# Autodesk Inventor assembly: CL4-100
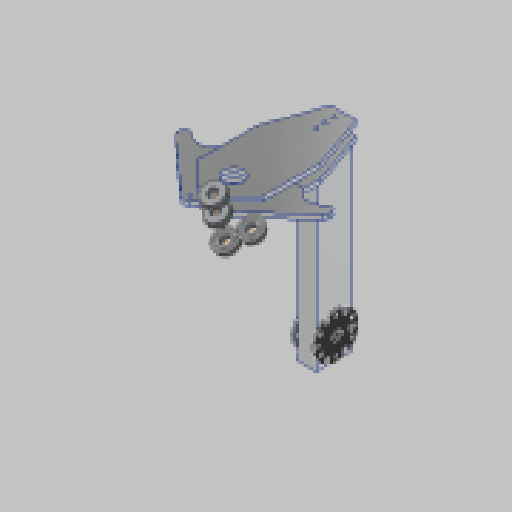
[picture p0: Inventor's stored thumbnail of the model, 512x512]
Saved by Autodesk Inventor 2023.5 (Build 275446000, 446)
## iProperties
Created: 2025-02-04
Part Number: CL4-100
Document SubType Name: Assembly
Designer: brand
Author: brand
## Documents named in this file (11)
- C:\Users\slick\OneDrive\Desktop\2025-ReefScape---CAD\Climber\CL4\CL4-100.iam
- C:\Users\slick\OneDrive\Desktop\2025-ReefScape---CAD\Climber\CL4\CL4-001.ipt
- C:\Users\slick\OneDrive\Desktop\2025-ReefScape---CAD\Climber\CL4\CL4-004.ipt
- C:\Users\slick\OneDrive\Desktop\2025-ReefScape---CAD\Field Items\Full Field\FE-2025\GE-25201.iam
- C:\Users\slick\OneDrive\Desktop\2025-ReefScape---CAD\Climber\CL4\02_Barb Assembly (1)\02_Barb Assembly (1).iam
- C:\Users\slick\OneDrive\Desktop\2025-ReefScape---CAD\Climber\CL4\CL4-005.ipt
- C:\Users\slick\OneDrive\Desktop\2025-ReefScape---CAD\Climber\CL4\CL4-006.ipt
- C:\Users\slick\OneDrive\Desktop\2025-ReefScape---CAD\COMMON PARTS\HUBS\WCP-1388.ipt
- C:\Users\slick\OneDrive\Desktop\2025-ReefScape---CAD\Climber\CL4\CL4-017.ipt
- C:\Users\slick\OneDrive\Desktop\2025-ReefScape---CAD\COMMON PARTS\BEARINGS\0_500_ID_x_1_125_OD_x_0_313_WD_Flanged_Bearing_217-2731.ipt
- C:\Users\slick\OneDrive\Desktop\2025-ReefScape---CAD\Climber\CL4\CL4-022.ipt
## Components (18 placed, 10 different names)
1. CL4-001:1 — Mate:7, Flush:6, Flush:7, Flush:8, Insert:2, Mate:14, Insert:3, Mate:15, Mate:16, Mate:17, Mate:20, Mate:21, Flush:10
2. CL4-005:1 — Flush:8, Flush:9, Mate:8, Mate:17, Insert:4, Insert:8, Insert:11
3. CL4-005:2 — Flush:9, Mate:8, Mate:9, Mate:12, Insert:1, Insert:7, Insert:14
4. CL4-004:1 — Mate:2, Mate:5, Mate:13, Mate:19, Insert:5
5. CL4-004:2 — Mate:2, Mate:5, Mate:9, Mate:12, Mate:13, Mate:18, Insert:6
6. GE-25201:1 [sub-assembly] — Mate:7
7. 02_Barb Assembly (1):1 [sub-assembly] — Flush:6, Flush:7
8. CL4-006:1 — Insert:1, Mate:18, Mate:19
9. WCP-1388:1 — Insert:2, Mate:14
10. WCP-1388:2 — Insert:3, Mate:15
11. CL4-017:1 — Mate:20, Mate:21, Flush:10
12. 0_500_ID_x_1_125_OD_x_0_313_WD_Flanged_Bearing_217-2731:1 — Insert:5, Mate:23
13. 0_500_ID_x_1_125_OD_x_0_313_WD_Flanged_Bearing_217-2731:2 — Insert:6, Mate:22
14. 0_500_ID_x_1_125_OD_x_0_313_WD_Flanged_Bearing_217-2731:3 — Insert:7, Mate:22
15. 0_500_ID_x_1_125_OD_x_0_313_WD_Flanged_Bearing_217-2731:4 — Insert:4, Mate:23
16. CL4-022:1 — Insert:8, Insert:9, Insert:11, Insert:12
17. CL4-022:2 — Insert:9, Insert:10, Insert:12, Insert:13
18. CL4-022:3 — Insert:10, Insert:13, Insert:14
## Relationships (37: Mate 17, Insert 14, Flush 6)
- Mate:2: CL4-004:1 ↔ CL4-004:2
- Mate:5: CL4-004:1 ↔ CL4-004:2
- [Flush]: CL4-001:1 ↔ CL4-005:1
- Mate:7: CL4-001:1 ↔ GE-25201:1
- Flush:6: CL4-001:1 ↔ 02_Barb Assembly (1):1
- Flush:7: CL4-001:1 ↔ 02_Barb Assembly (1):1
- Flush:8: CL4-001:1 ↔ CL4-005:1
- Flush:9: CL4-005:1 ↔ CL4-005:2
- Mate:8: CL4-005:1 ↔ CL4-005:2
- Mate:9: CL4-005:2 ↔ CL4-004:2
- Mate:12: CL4-005:2 ↔ CL4-004:2
- Mate:13: CL4-004:1 ↔ CL4-004:2
- Insert:1: CL4-005:2 ↔ CL4-006:1
- Insert:2: CL4-001:1 ↔ WCP-1388:1
- Mate:14: CL4-001:1 ↔ WCP-1388:1
- Insert:3: CL4-001:1 ↔ WCP-1388:2
- Mate:15: CL4-001:1 ↔ WCP-1388:2
- Mate:16: CL4-001:1
- Mate:17: CL4-001:1 ↔ CL4-005:1
- Mate:18: CL4-004:2 ↔ CL4-006:1
- Mate:19: CL4-004:1 ↔ CL4-006:1
- Mate:20: CL4-001:1 ↔ CL4-017:1
- Mate:21: CL4-001:1 ↔ CL4-017:1
- Flush:10: CL4-001:1 ↔ CL4-017:1
- Insert:4: CL4-005:1 ↔ 0_500_ID_x_1_125_OD_x_0_313_WD_Flanged_Bearing_217-2731:4
- Insert:5: CL4-004:1 ↔ 0_500_ID_x_1_125_OD_x_0_313_WD_Flanged_Bearing_217-2731:1
- Insert:6: CL4-004:2 ↔ 0_500_ID_x_1_125_OD_x_0_313_WD_Flanged_Bearing_217-2731:2
- Insert:7: CL4-005:2 ↔ 0_500_ID_x_1_125_OD_x_0_313_WD_Flanged_Bearing_217-2731:3
- Mate:22: 0_500_ID_x_1_125_OD_x_0_313_WD_Flanged_Bearing_217-2731:2 ↔ 0_500_ID_x_1_125_OD_x_0_313_WD_Flanged_Bearing_217-2731:3
- Mate:23: 0_500_ID_x_1_125_OD_x_0_313_WD_Flanged_Bearing_217-2731:1 ↔ 0_500_ID_x_1_125_OD_x_0_313_WD_Flanged_Bearing_217-2731:4
- Insert:8: CL4-005:1 ↔ CL4-022:1
- Insert:9: CL4-022:1 ↔ CL4-022:2
- Insert:10: CL4-022:2 ↔ CL4-022:3
- Insert:11: CL4-005:1 ↔ CL4-022:1
- Insert:12: CL4-022:1 ↔ CL4-022:2
- Insert:13: CL4-022:2 ↔ CL4-022:3
- Insert:14: CL4-005:2 ↔ CL4-022:3
